# Autodesk Inventor assembly: Shooting Mechanism Assembly.final
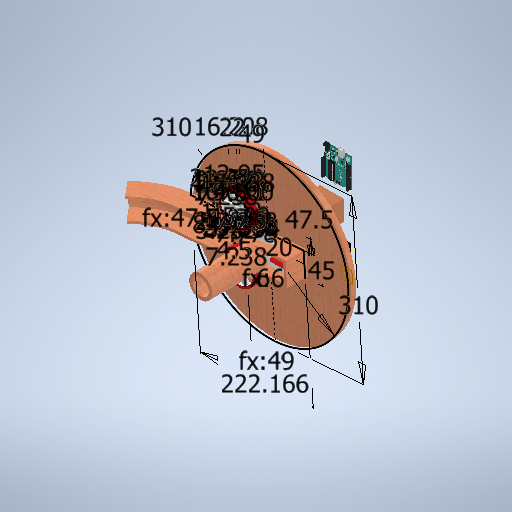
[picture p0: Inventor's stored thumbnail of the model, 512x512]
Saved by Autodesk Inventor 2025.2 (Build 292293000, 293)
## iProperties
Created: 2026-04-11
Part Number: Shooting Mechanism Assembly.final
Document SubType Name: Assembly
Designer: abdul
Author: abdul
## Documents named in this file (11)
- D:\Semester 2\Basics of Mechatronics\BO\Shooting Mechanism Assembly.final.iam
- D:\Semester 2\Basics of Mechatronics\BO\Assembly1.iam
- D:\Semester 2\Basics of Mechatronics\BO\Rotating Base.ipt
- D:\Semester 2\Basics of Mechatronics\BO\Servo Mount.ipt
- D:\Semester 2\Basics of Mechatronics\BO\Servo Stand.ipt
- D:\Semester 2\Basics of Mechatronics\BO\MG_996R.iam
- D:\Semester 2\Basics of Mechatronics\BO\flywheel.ipt
- D:\Semester 2\Basics of Mechatronics\BO\H-brug.ipt
- D:\Semester 2\Basics of Mechatronics\BO\arduinouno.ipt
- D:\Semester 2\Basics of Mechatronics\BO\Shooting Ramp.ipt
- D:\Semester 2\Basics of Mechatronics\BO\Mini Push Pull Solenoid 4mm.ipt
## Components (12 placed, 10 different names)
1. Servo Mount:3 — Mate:20, Mate:21, Mate:22, Mate:23, Mate:24, Mate:25
2. Servo Stand:4 — Mate:20, Mate:21, Mate:22
3. MG_996R:1 [sub-assembly] — Mate:23, Mate:24, Mate:25, Mate:40
4. flywheel:1 — Mate:31, Mate:32, Mate:59
5. flywheel:2 — Mate:30, Mate:33, Mate:60
6. Rotating Base:1 — Mate:26, Mate:27, Mate:28, Mate:29, Mate:34, Mate:35, Mate:40, Mate:42, Mate:43, Mate:44
7. Assembly1:1 [sub-assembly] — Mate:26, Mate:29, Mate:30, Mate:33, Mate:35, Mate:60
8. Assembly1:2 [sub-assembly] — Mate:27, Mate:28, Mate:31, Mate:32, Mate:34, Mate:59
9. H-brug:1
10. arduinouno:1
11. Shooting Ramp:1 — Mate:42, Mate:43, Mate:44, Mate:56, Mate:57
12. Mini Push Pull Solenoid 4mm:1 — Mate:56, Mate:57
## Relationships (24: Mate 24)
- Mate:20: Servo Mount:3 ↔ Servo Stand:4
- Mate:21: Servo Mount:3 ↔ Servo Stand:4
- Mate:22: Servo Mount:3 ↔ Servo Stand:4
- Mate:23: Servo Mount:3 ↔ MG_996R:1
- Mate:24: Servo Mount:3 ↔ MG_996R:1
- Mate:25: Servo Mount:3 ↔ MG_996R:1
- Mate:26: Rotating Base:1 ↔ Assembly1:1
- Mate:27: Rotating Base:1 ↔ Assembly1:2
- Mate:28: Rotating Base:1 ↔ Assembly1:2
- Mate:29: Rotating Base:1 ↔ Assembly1:1
- Mate:30: flywheel:2 ↔ Assembly1:1
- Mate:31: flywheel:1 ↔ Assembly1:2
- Mate:32: flywheel:1 ↔ Assembly1:2
- Mate:33: flywheel:2 ↔ Assembly1:1
- Mate:34: Rotating Base:1 ↔ Assembly1:2
- Mate:35: Rotating Base:1 ↔ Assembly1:1
- Mate:40: MG_996R:1 ↔ Rotating Base:1
- Mate:42: Rotating Base:1 ↔ Shooting Ramp:1
- Mate:43: Rotating Base:1 ↔ Shooting Ramp:1
- Mate:44: Rotating Base:1 ↔ Shooting Ramp:1
- Mate:56 (100 mm): Shooting Ramp:1 ↔ Mini Push Pull Solenoid 4mm:1
- Mate:57 (5 mm): Shooting Ramp:1 ↔ Mini Push Pull Solenoid 4mm:1
- Mate:59: flywheel:1 ↔ Assembly1:2
- Mate:60: flywheel:2 ↔ Assembly1:1
## Named parameters: Finish1_Area = 751.824, Finish2_Area = 15.835, Finish3_Area = 147.788, Finish4_Area = 25.6198, Finish5_Area = 70.7173
note: some values were not read from the file. Shown as the stored number, unit unknown: "Finish1_Area", "Finish2_Area", "Finish3_Area", "Finish4_Area", "Finish5_Area".
